# Autodesk Inventor assembly: Gearmotor
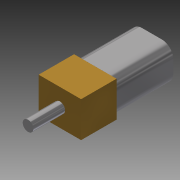
[picture p0: Inventor's stored thumbnail of the model, 180x180]
Saved by Autodesk Inventor 2013 (Build 170138000, 138)
## iProperties
Created: 2015-07-02
Part Number: Gearmotor
Document SubType Name: Assembly
Designer: Kyle
Mass: 9.38144 g
Surface Area: 27.0215 cm^2
Volume: 1.12155 cm^3
Density: 8.36474 g/cm^3
Author: Kyle
## Documents named in this file (4)
- C:\Users\Kyle\Documents\Project documentation\Combat Robot\CAD\V1.0\Gearmotor.iam
- C:\Users\Kyle\Documents\Project documentation\Combat Robot\CAD\V1.0\Gearmotor_Motor.ipt
- C:\Users\Kyle\Documents\Project documentation\Combat Robot\CAD\V1.0\Gearmotor_Gear.ipt
- C:\Users\Kyle\Documents\Project documentation\Combat Robot\CAD\V1.0\Gearmotor_Shaft.ipt
## Components (3 placed, 3 different names)
1. Gearmotor_Motor:1 — Mate:1, Flush:1, Flush:2
2. Gearmotor_Gear:1 — Mate:1, Flush:1, Flush:2, Mate:2, Mate:3, Mate:4
3. Gearmotor_Shaft:1 — Mate:2, Mate:3, Mate:4
## Relationships (6: Mate 4, Flush 2)
- Mate:1: Gearmotor_Motor:1 ↔ Gearmotor_Gear:1
- Flush:1: Gearmotor_Motor:1 ↔ Gearmotor_Gear:1
- Flush:2: Gearmotor_Motor:1 ↔ Gearmotor_Gear:1
- Mate:2: Gearmotor_Gear:1 ↔ Gearmotor_Shaft:1
- Mate:3 (-5.9944 mm): Gearmotor_Gear:1 ↔ Gearmotor_Shaft:1
- Mate:4 (-5.0038 mm): Gearmotor_Gear:1 ↔ Gearmotor_Shaft:1
